# Autodesk Inventor assembly: czlon 1 i 2
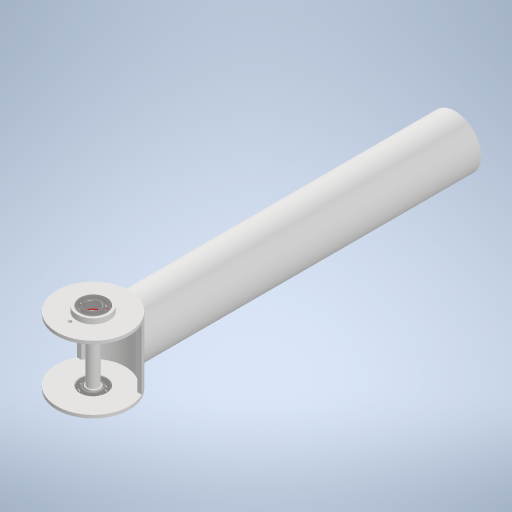
[picture p0: Inventor's stored thumbnail of the model, 512x512]
Saved by Autodesk Inventor 2023 (Build 270158000, 158)
## iProperties
Created: 2023-04-09
Part Number: czlon 1 i 2
Document SubType Name: Assembly
Designer: Wiktor
Author: Wiktor
## Documents named in this file (4)
- C:\Users\Wiktor\Documents\Manipulator\czlon 1 i 2.iam
- C:\Users\Wiktor\Documents\Manipulator\czlon i przekladnia.iam
- C:\Users\Wiktor\Documents\Manipulator\czlon 1 i 2\Design Accelerator\Łożysko1.iam
- C:\Users\Wiktor\Documents\Manipulator\wal_czlon_2.ipt
## Components (4 placed, 3 different names)
1. czlon i przekladnia:1 [sub-assembly] — Zestawiające:1, Zestawiające:2, Zestawiające:3, Zestawiające:4, Zestawiające:5, Zestawiające:6, Zestawiające:7
2. Łożysko:1 [sub-assembly] — Zestawiające:1, Zestawiające:2
3. Łożysko:3 [sub-assembly] — Zestawiające:3, Zestawiające:4, Zestawiające:5
4. wal_czlon_2:1 — Zestawiające:6, Zestawiające:7
## Relationships (7: Mate 7)
- Zestawiające:1 [Mate]: czlon i przekladnia:1 ↔ Łożysko:1
- Zestawiające:2 [Mate]: czlon i przekladnia:1 ↔ Łożysko:1
- Zestawiające:3 [Mate]: czlon i przekladnia:1 ↔ Łożysko:3
- Zestawiające:4 [Mate]: czlon i przekladnia:1 ↔ Łożysko:3
- Zestawiające:5 [Mate]: czlon i przekladnia:1 ↔ Łożysko:3
- Zestawiające:6 [Mate]: czlon i przekladnia:1 ↔ wal_czlon_2:1
- Zestawiające:7 [Mate]: czlon i przekladnia:1 ↔ wal_czlon_2:1
